# Autodesk Inventor assembly: JH_Greifer_Scheibe
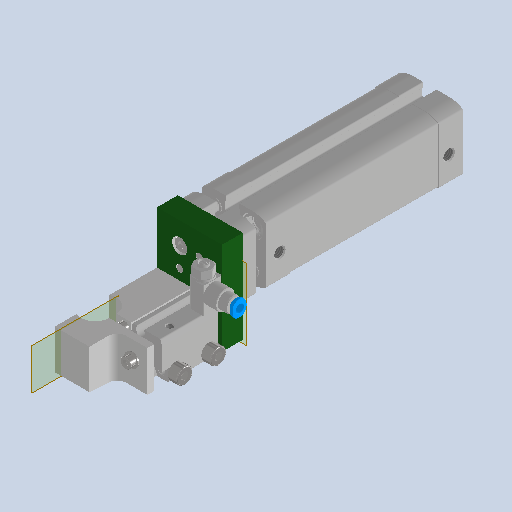
[picture p0: Inventor's stored thumbnail of the model, 512x512]
Saved by Autodesk Inventor 2025.2 (Build 292293000, 293)
## iProperties
Created: 2025-06-16
Part Number: JH_Greifer_Scheibe
Document SubType Name: Assembly
Designer: Jakob
Author: Jakob
## Documents named in this file (16)
- C:\Users\tino\Documents_VM\Konstruieren_CAD\Useless Box\Eigene Bauteile\JH_Greifer_Unterlegscheibe\Eigene Bauteile\JH_Greifer_Scheibe.iam
- C:\Users\tino\Documents_VM\Konstruieren_CAD\Useless Box\Eigene Bauteile\JH_Greifer_Unterlegscheibe\Eigene Bauteile\JH_int_Greiferkoerper.ipt
- C:\Users\tino\Documents_VM\Konstruieren_CAD\Useless Box\Eigene Bauteile\JH_Greifer_Unterlegscheibe\Eigene Bauteile\JH_int_Greiferkoerper_Gegenstueck.ipt
- C:\Users\tino\Documents_VM\Konstruieren_CAD\Useless Box\Eigene Bauteile\JH_Greifer_Unterlegscheibe\Kaufteile\AIS2024\5267300 AEN-S-6-5-I-A---(0_high).iam
- C:\Users\tino\Documents_VM\Konstruieren_CAD\Useless Box\Standart Bauteile\DIN 125 - A 2,7.ipt
- C:\Users\tino\Documents_VM\Konstruieren_CAD\Useless Box\Standart Bauteile\DIN EN ISO 4762 - M2,5 x 5.ipt
- C:\Users\tino\Documents_VM\Konstruieren_CAD\Useless Box\Standart Bauteile\DIN EN ISO 2338 - 4 h8 x 14.ipt
- C:\Users\tino\Documents_VM\Konstruieren_CAD\Useless Box\Eigene Bauteile\JH_Greifer_Unterlegscheibe\Kaufteile\AIS2024\Unterlegscheibe.ipt
- C:\Users\tino\Documents_VM\Konstruieren_CAD\Useless Box\Eigene Bauteile\JH_Greifer_Unterlegscheibe\Kaufteile\Drosselrückschlagventil\175043 GRLZ-M3-QS-3.ipt
- C:\Users\tino\Documents_VM\Konstruieren_CAD\Useless Box\Standart Bauteile\DIN EN ISO 4762 - M4 x 16.ipt
- C:\Users\tino\Documents_VM\Konstruieren_CAD\Useless Box\Eigene Bauteile\JH_Greifer_Unterlegscheibe\Kaufteile\Führungszylinder\AIS2024\537123 ADNGF-12-50-P-A---(0).iam
- C:\Users\tino\Documents_VM\Konstruieren_CAD\Useless Box\Eigene Bauteile\JH_Greifer_Unterlegscheibe\Eigene Bauteile\JH_int_Adapterplatte.ipt
- C:\Users\tino\Documents_VM\Konstruieren_CAD\Useless Box\Standart Bauteile\DIN EN ISO 4762 - M3 x 5.ipt
- C:\Users\tino\Documents_VM\Konstruieren_CAD\Useless Box\Standart Bauteile\DIN EN ISO 2338 - 3 h8 x 10.ipt
- C:\Users\tino\Documents_VM\Konstruieren_CAD\Useless Box\Standart Bauteile\DIN EN ISO 2338 - 3 h8 x 14.ipt
- C:\Users\tino\Documents_VM\Konstruieren_CAD\Useless Box\Standart Bauteile\DIN EN ISO 4762 - M3 x 10.ipt
## Components (20 placed, 15 different names)
1. JH_int_Greiferkoerper:1 — Fluchtend:1, Fluchtend:2, Fluchtend:3, Passend:2, Passend:3, Passend:4, Passend:9, Passend:10, Passend:11, Passend:12, Passend:28, Passend:29, Passend:30
2. JH_int_Greiferkoerper_Gegenstueck:1 — Passend:1, Fluchtend:4, Fluchtend:5, Passend:5, Fluchtend:6, Passend:20
3. 5267300 AEN-S-6-5-I-A---(0_high):1 [sub-assembly] — Passend:2, Passend:3, Passend:4, Fluchtend:5, Passend:6, Passend:7, Passend:18, Passend:19, Passend:24, Passend:25, Passend:26, Passend:27
4. DIN 125 - A 2,7:1 — Passend:5, Passend:6, Passend:8
5. DIN EN ISO 4762 - M2,5 x 5:1 — Passend:7, Passend:8
6. DIN EN ISO 2338 - 4 h8 x 14:1 — Passend:9, Passend:10
7. DIN EN ISO 2338 - 4 h8 x 14:2 — Passend:11, Passend:12
8. DIN 9021 2,7:1 — Passend:20
9. 175043 GRLZ-M3-QS-3:1 — Winkel:1, Passend:18, Passend:19
10. DIN EN ISO 4762 - M4 x 16:1 — Passend:24, Passend:27
11. DIN EN ISO 4762 - M4 x 16:2 — Passend:25, Passend:26
12. 537123 ADNGF-12-50-P-A---(0):1 [sub-assembly] — Passend:31, Passend:32, Passend:33
13. JH_int_Adapterplatte:1 — Passend:28, Passend:29, Passend:30, Passend:31, Passend:32, Passend:33, Passend:34, Passend:35, Passend:36, Passend:37, Passend:38, Fluchtend:7, Passend:39, Passend:40, Fluchtend:8, Fluchtend:9, Passend:41, Passend:42, Passend:43, Passend:44
14. DIN EN ISO 4762 - M3 x 5:1 — Passend:34, Passend:36
15. DIN EN ISO 4762 - M3 x 5:2 — Passend:35, Passend:37
16. DIN EN ISO 2338 - 3 h8 x 10:1 — Passend:38, Fluchtend:7
17. DIN EN ISO 2338 - 3 h8 x 14:1 — Passend:40, Fluchtend:8
18. DIN EN ISO 2338 - 3 h8 x 14:2 — Passend:39, Fluchtend:9
19. DIN EN ISO 4762 - M3 x 10:1 — Passend:42, Passend:44
20. DIN EN ISO 4762 - M3 x 10:2 — Passend:41, Passend:43
## Relationships (46: Mate 36, Flush 9, Angle 1)
- Fluchtend:1 [Flush]: JH_int_Greiferkoerper:1
- Fluchtend:2 [Flush]: JH_int_Greiferkoerper:1
- Fluchtend:3 [Flush]: JH_int_Greiferkoerper:1
- Passend:1 [Mate]: JH_int_Greiferkoerper_Gegenstueck:1
- Fluchtend:4 [Flush]: JH_int_Greiferkoerper_Gegenstueck:1
- Passend:2 [Mate]: JH_int_Greiferkoerper:1 ↔ 5267300 AEN-S-6-5-I-A---(0_high):1
- Passend:3 [Mate]: JH_int_Greiferkoerper:1 ↔ 5267300 AEN-S-6-5-I-A---(0_high):1
- Passend:4 [Mate]: JH_int_Greiferkoerper:1 ↔ 5267300 AEN-S-6-5-I-A---(0_high):1
- Fluchtend:5 [Flush]: JH_int_Greiferkoerper_Gegenstueck:1 ↔ 5267300 AEN-S-6-5-I-A---(0_high):1
- Passend:5 [Mate]: JH_int_Greiferkoerper_Gegenstueck:1 ↔ DIN 125 - A 2,7:1
- Passend:6 [Mate]: 5267300 AEN-S-6-5-I-A---(0_high):1 ↔ DIN 125 - A 2,7:1
- Passend:7 [Mate]: 5267300 AEN-S-6-5-I-A---(0_high):1 ↔ DIN EN ISO 4762 - M2,5 x 5:1
- Passend:8 [Mate]: DIN 125 - A 2,7:1 ↔ DIN EN ISO 4762 - M2,5 x 5:1
- Passend:9 [Mate]: JH_int_Greiferkoerper:1 ↔ DIN EN ISO 2338 - 4 h8 x 14:1
- Passend:10 [Mate]: JH_int_Greiferkoerper:1 ↔ DIN EN ISO 2338 - 4 h8 x 14:1
- Passend:11 [Mate]: JH_int_Greiferkoerper:1 ↔ DIN EN ISO 2338 - 4 h8 x 14:2
- Passend:12 [Mate]: JH_int_Greiferkoerper:1 ↔ DIN EN ISO 2338 - 4 h8 x 14:2
- Winkel:1 [Angle] (0 deg): 175043 GRLZ-M3-QS-3:1
- Passend:18 [Mate]: 5267300 AEN-S-6-5-I-A---(0_high):1 ↔ 175043 GRLZ-M3-QS-3:1
- Passend:19 [Mate]: 5267300 AEN-S-6-5-I-A---(0_high):1 ↔ 175043 GRLZ-M3-QS-3:1
- Fluchtend:6 [Flush] (-2.541 mm): JH_int_Greiferkoerper_Gegenstueck:1
- Passend:20 [Mate] (7.95 mm): JH_int_Greiferkoerper_Gegenstueck:1 ↔ DIN 9021 2,7:1
- Passend:24 [Mate]: 5267300 AEN-S-6-5-I-A---(0_high):1 ↔ DIN EN ISO 4762 - M4 x 16:1
- Passend:25 [Mate]: 5267300 AEN-S-6-5-I-A---(0_high):1 ↔ DIN EN ISO 4762 - M4 x 16:2
- Passend:26 [Mate]: 5267300 AEN-S-6-5-I-A---(0_high):1 ↔ DIN EN ISO 4762 - M4 x 16:2
- Passend:27 [Mate]: 5267300 AEN-S-6-5-I-A---(0_high):1 ↔ DIN EN ISO 4762 - M4 x 16:1
- Passend:28 [Mate]: JH_int_Greiferkoerper:1 ↔ JH_int_Adapterplatte:1
- Passend:29 [Mate]: JH_int_Greiferkoerper:1 ↔ JH_int_Adapterplatte:1
- Passend:30 [Mate]: JH_int_Greiferkoerper:1 ↔ JH_int_Adapterplatte:1
- Passend:31 [Mate]: 537123 ADNGF-12-50-P-A---(0):1 ↔ JH_int_Adapterplatte:1
- Passend:32 [Mate]: 537123 ADNGF-12-50-P-A---(0):1 ↔ JH_int_Adapterplatte:1
- Passend:33 [Mate]: 537123 ADNGF-12-50-P-A---(0):1 ↔ JH_int_Adapterplatte:1
- Passend:34 [Mate]: JH_int_Adapterplatte:1 ↔ DIN EN ISO 4762 - M3 x 5:1
- Passend:35 [Mate]: JH_int_Adapterplatte:1 ↔ DIN EN ISO 4762 - M3 x 5:2
- Passend:36 [Mate]: JH_int_Adapterplatte:1 ↔ DIN EN ISO 4762 - M3 x 5:1
- Passend:37 [Mate]: JH_int_Adapterplatte:1 ↔ DIN EN ISO 4762 - M3 x 5:2
- Passend:38 [Mate]: JH_int_Adapterplatte:1 ↔ DIN EN ISO 2338 - 3 h8 x 10:1
- Fluchtend:7 [Flush]: JH_int_Adapterplatte:1 ↔ DIN EN ISO 2338 - 3 h8 x 10:1
- Passend:39 [Mate]: JH_int_Adapterplatte:1 ↔ DIN EN ISO 2338 - 3 h8 x 14:2
- Passend:40 [Mate]: JH_int_Adapterplatte:1 ↔ DIN EN ISO 2338 - 3 h8 x 14:1
- Fluchtend:8 [Flush]: JH_int_Adapterplatte:1 ↔ DIN EN ISO 2338 - 3 h8 x 14:1
- Fluchtend:9 [Flush]: JH_int_Adapterplatte:1 ↔ DIN EN ISO 2338 - 3 h8 x 14:2
- Passend:41 [Mate]: JH_int_Adapterplatte:1 ↔ DIN EN ISO 4762 - M3 x 10:2
- Passend:42 [Mate]: JH_int_Adapterplatte:1 ↔ DIN EN ISO 4762 - M3 x 10:1
- Passend:43 [Mate]: JH_int_Adapterplatte:1 ↔ DIN EN ISO 4762 - M3 x 10:2
- Passend:44 [Mate]: JH_int_Adapterplatte:1 ↔ DIN EN ISO 4762 - M3 x 10:1
